# Autodesk Inventor assembly: Custom Vice V1
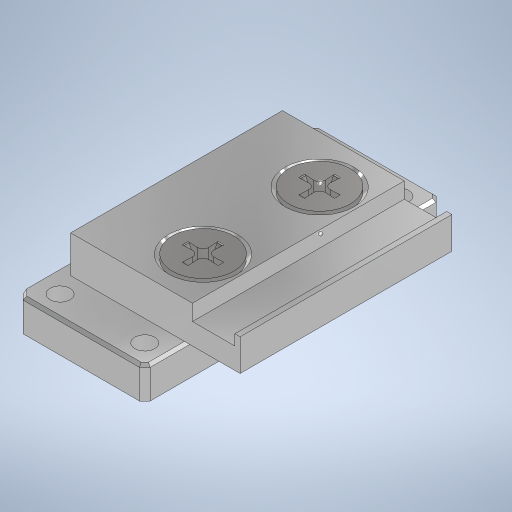
[picture p0: Inventor's stored thumbnail of the model, 512x512]
Saved by Autodesk Inventor 2023.2 (Build 272271000, 271)
## iProperties
Created: 2024-03-01
Part Number: Custom Vice V1
Document SubType Name: Assembly
Designer: Nathan Cai
Author: Nathan Cai
## Documents named in this file (4)
- E:\Documents\Inventor\Custom Vice V1\Custom Vice V1.iam
- E:\Documents\Inventor\Custom Vice V1\Base - Stationary.ipt
- E:\Documents\Inventor\Custom Vice V1\Jaw.ipt
- E:\Documents\Inventor\Content Center Files\R2023\en-US\ANSI B18.6.3(12)\ANSI B18.6.3 - 7_16-14 UNC - 0.75(15_).ipt
## Components (4 placed, 3 different names)
1. Base - Stationary:1 — Mate:1, Mate:2, Mate:3
2. Jaw:1 — Mate:1, Mate:2, Mate:3, Mate:4, Mate:5
3. Cross Recessed Flat Countersunk Head Machine Screw - Type I - Inch 7/16-14 x 3/4:1 — Mate:4
4. Cross Recessed Flat Countersunk Head Machine Screw - Type I - Inch 7/16-14 x 3/4:2 — Mate:5
## Relationships (5: Mate 5)
- Mate:1: Base - Stationary:1 ↔ Jaw:1
- Mate:2: Base - Stationary:1 ↔ Jaw:1
- Mate:3: Base - Stationary:1 ↔ Jaw:1
- Mate:4: Jaw:1 ↔ Cross Recessed Flat Countersunk Head Machine Screw - Type I - Inch 7/16-14 x 3/4:1
- Mate:5: Jaw:1 ↔ Cross Recessed Flat Countersunk Head Machine Screw - Type I - Inch 7/16-14 x 3/4:2
